# Autodesk Inventor assembly: Assembly
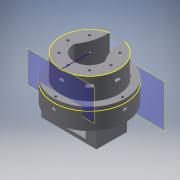
[picture p0: Inventor's stored thumbnail of the model, 180x180]
Saved by Autodesk Inventor 2017 (Build 210142000, 142)
## iProperties
Created: 2017-08-04
Part Number: Assembly
Document SubType Name: Assembly
Designer: Bardo91
Author: Bardo91
## Documents named in this file (4)
- D:\programming\cad_hexacopter\arm_3dog\Assembly.iam
- D:\programming\cad_hexacopter\arm_3dog\Base.ipt
- D:\programming\cad_hexacopter\arm_3dog\rotBase.ipt
- D:\programming\cad_hexacopter\arm_3dog\rotBaseServo.ipt
## Components (3 placed, 3 different names)
1. Base:1 — Mate:1, Mate:4
2. rotBase:1 — Mate:2, Mate:3, Mate:4
3. rotBaseServo:1 — Mate:1, Mate:2, Mate:3
## Relationships (4: Mate 4)
- Mate:1: Base:1 ↔ rotBaseServo:1
- Mate:2: rotBase:1 ↔ rotBaseServo:1
- Mate:3: rotBase:1 ↔ rotBaseServo:1
- Mate:4: Base:1 ↔ rotBase:1
